# Autodesk Inventor assembly: LCD Mount Front
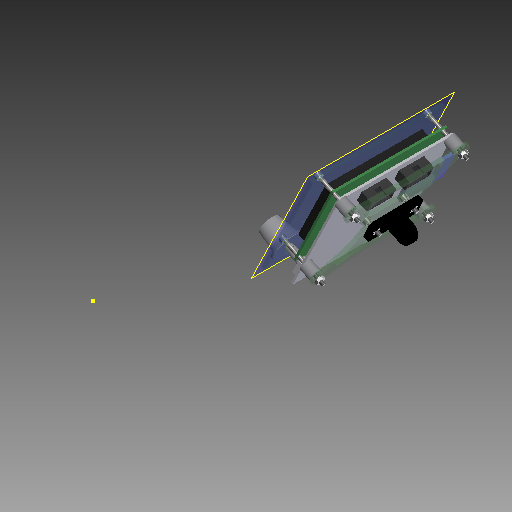
[picture p0: Inventor's stored thumbnail of the model, 512x512]
Saved by Autodesk Inventor 2017 (Build 210142000, 142)
## iProperties
Created: 2016-08-23
Part Number: LCD Mount Front
Document SubType Name: Assembly
Designer: User
Author: User
## Documents named in this file (9)
- C:\All INVENTOR\SL-Inventor\SL-Beast 3D Printer\LCD Mount Front.iam
- C:\All INVENTOR\SL-Inventor\SL-Beast 3D Printer\Smart-ControllerandBracket.iam
- C:\All INVENTOR\SL-Inventor\SL-Beast 3D Printer\en-US\ANSI B18.3.1M(6)\ANSI B18.3.1M - M3x0.5 x 10(1).ipt
- C:\All INVENTOR\SL-Inventor\SL-Beast 3D Printer\en-US\CSN EN 24 036\CSN EN 24 036 - M3.ipt
- C:\All INVENTOR\SL-Inventor\SL-Beast 3D Printer\Knob.ipt
- C:\All INVENTOR\SL-Inventor\SL-Beast 3D Printer\LCD-Front.ipt
- C:\All INVENTOR\SL-Inventor\SL-Beast 3D Printer\LCD Back.ipt
- C:\All INVENTOR\SL-Inventor\SL-Beast 3D Printer\LCD-Spacer.ipt
- C:\All INVENTOR\SL-Inventor\SL-Beast 3D Printer\LCD Mount Part 3 side.ipt
## Components (13 placed, 8 different names)
1. Smart-ControllerandBracket:1 [sub-assembly] — Mate:15, Angle:1
2. Forged Socket Head Cap Screw - Metric M3x0.5 x 10:1
3. CSN EN 24036 M3:1
4. Knob:1
5. LCD-Front:1 — Mate:15, Angle:1
6. LCD Back:1
7. LCD-Spacer:1
8. LCD-Spacer:2
9. LCD-Spacer:3
10. LCD-Spacer:4
11. Forged Socket Head Cap Screw - Metric M3x0.5 x 10:2
12. CSN EN 24036 M3:2
13. LCD Mount Part 3 side:1
## Relationships (19: Mate 14, Flush 4, Angle 1)
- [Mate]: Forged Socket Head Cap Screw - Metric M3x0.5 x 10:1 ↔ CSN EN 24036 M3:1
- [Mate]: Smart-ControllerandBracket:1 ↔ LCD-Spacer:1
- [Mate]: Smart-ControllerandBracket:1 ↔ LCD-Spacer:2
- [Mate]: Smart-ControllerandBracket:1 ↔ LCD-Spacer:3
- [Mate]: Smart-ControllerandBracket:1 ↔ LCD-Spacer:4
- [Flush]: LCD-Spacer:3 ↔ LCD-Spacer:4
- [Flush]: LCD-Spacer:1 ↔ LCD-Spacer:3
- [Flush]: LCD-Spacer:1 ↔ LCD-Spacer:2
- [Mate]: Smart-ControllerandBracket:1 ↔ LCD-Spacer:2
- [Mate]: LCD Back:1 ↔ LCD-Spacer:1
- [Mate]: Forged Socket Head Cap Screw - Metric M3x0.5 x 10:2 ↔ CSN EN 24036 M3:2
- [Mate]: LCD Back:1 ↔ Forged Socket Head Cap Screw - Metric M3x0.5 x 10:2
- [Mate]: Forged Socket Head Cap Screw - Metric M3x0.5 x 10:2 ↔ CSN EN 24036 M3:2
- [Flush]: CSN EN 24036 M3:1 ↔ CSN EN 24036 M3:2
- [Mate]: Forged Socket Head Cap Screw - Metric M3x0.5 x 10:1 ↔ LCD Mount Part 3 side:1
- [Mate]: Forged Socket Head Cap Screw - Metric M3x0.5 x 10:2 ↔ LCD Mount Part 3 side:1
- [Mate]: LCD Back:1 ↔ LCD Mount Part 3 side:1
- Mate:15: Smart-ControllerandBracket:1 ↔ LCD-Front:1
- Angle:1 (0 deg): Smart-ControllerandBracket:1 ↔ LCD-Front:1
## Named parameters: d71_d45 = 0 mm
